# Autodesk Inventor assembly: item_Handgriff_PA120_Assembly
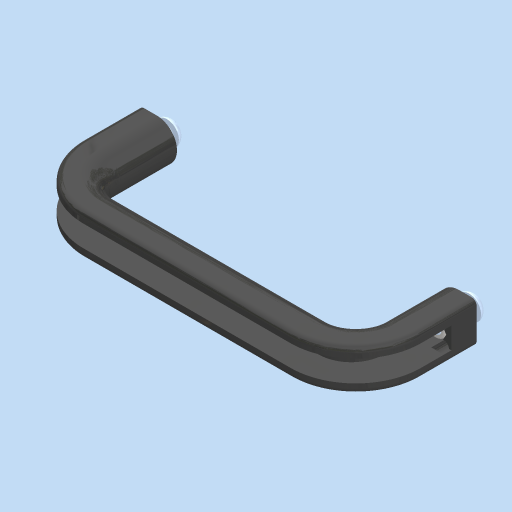
[picture p0: Inventor's stored thumbnail of the model, 512x512]
Saved by Autodesk Inventor 2023.2 (Build 272271000, 271)
## iProperties
Created: 2024-01-15
Part Number: item_Handgriff_PA120_Assembly
Document SubType Name: Assembly
Designer: Nils Bade
Author: Nils Bade
## Documents named in this file (5)
- C:\Users\nilsb\Documents\Inventor\Projektarbeit-Bade\Enclosure\item_Handgriff_PA120_Assembly.iam
- C:\Users\nilsb\Documents\Inventor\Projektarbeit-Bade\Enclosure\item_Handgriff PA 120.ipt
- C:\Users\nilsb\Documents\Inventor\Projektarbeit-Bade\RatRig_Standards\Hex Locking Nut - M5 v2.ipt
- C:\Users\nilsb\Documents\Inventor\Projektarbeit-Bade\Schrauben\item_Halbrundschraube M5x14_0041730.ipt
- item_Halbrundschraube M5x14_0041730.ipt
## Components (5 placed, 3 different names)
1. item_Handgriff PA 120:1 — Passend:1, Passend:2, Winkel:1, Winkel:2, Passend:3, Passend:4, Passend:5, Passend:6, Passend:7, Passend:8
2. Hex Locking Nut - M5 v2:1 — Passend:1, Winkel:2, Passend:3
3. Hex Locking Nut - M5 v2:2 — Passend:2, Winkel:1, Passend:4
4. item_Halbrundschraube M5x14_0041730:1 — Passend:5, Passend:8
5. item_Halbrundschraube M5x14_0041730:2 — Passend:6, Passend:7
## Relationships (10: Mate 8, Angle 2)
- Passend:1 [Mate]: item_Handgriff PA 120:1 ↔ Hex Locking Nut - M5 v2:1
- Passend:2 [Mate]: item_Handgriff PA 120:1 ↔ Hex Locking Nut - M5 v2:2
- Winkel:1 [Angle] (0 deg): item_Handgriff PA 120:1 ↔ Hex Locking Nut - M5 v2:2
- Winkel:2 [Angle] (0 deg): item_Handgriff PA 120:1 ↔ Hex Locking Nut - M5 v2:1
- Passend:3 [Mate]: item_Handgriff PA 120:1 ↔ Hex Locking Nut - M5 v2:1
- Passend:4 [Mate]: item_Handgriff PA 120:1 ↔ Hex Locking Nut - M5 v2:2
- Passend:5 [Mate]: item_Handgriff PA 120:1 ↔ item_Halbrundschraube M5x14_0041730:1
- Passend:6 [Mate]: item_Handgriff PA 120:1 ↔ item_Halbrundschraube M5x14_0041730:2
- Passend:7 [Mate] (4 mm): item_Handgriff PA 120:1 ↔ item_Halbrundschraube M5x14_0041730:2
- Passend:8 [Mate] (4 mm): item_Handgriff PA 120:1 ↔ item_Halbrundschraube M5x14_0041730:1
